# Autodesk Inventor assembly: XCarriageJHead
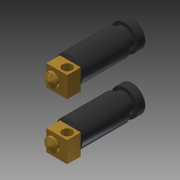
[picture p0: Inventor's stored thumbnail of the model, 180x180]
Saved by Autodesk Inventor 2015 (Build 190159000, 159)
## iProperties
Created: 2014-10-05
Part Number: XCarriageJHead
Document SubType Name: Assembly
Designer: Jack
Author: Jack
## Documents named in this file (2)
- C:\Users\Jack\ownCloud\Projects\CoreXY\InventorModel\XAxis\XCarriageJHead.iam
- C:\Users\Jack\ownCloud\Projects\CoreXY\InventorModel\HotEnds\JHeadmkV\JHeadmkV.iam
## Components (2 placed, 1 different names)
1. JHeadmkV:1 [sub-assembly] — Flush:1, Flush:2, Flush:3, Mate:1, Mate:2
2. JHeadmkV:2 [sub-assembly] — Flush:1, Flush:2
## Relationships (5: Flush 3, Mate 2)
- Flush:1: JHeadmkV:1 ↔ JHeadmkV:2
- Flush:2: JHeadmkV:1 ↔ JHeadmkV:2
- Flush:3: JHeadmkV:1
- Mate:1: JHeadmkV:1
- Mate:2: JHeadmkV:1
